# Autodesk Inventor assembly: CentralBeam1of2WithSails
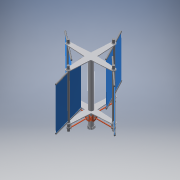
[picture p0: Inventor's stored thumbnail of the model, 180x180]
Saved by Autodesk Inventor 2016 SP1 (Build 200210100, 210)
## iProperties
Created: 2016-07-04
Part Number: CentralBeam1of2WithSails
Document SubType Name: Assembly
Designer: Tore Den Store
Author: Tore Den Store
## Documents named in this file (4)
- C:\Users\Jonatan\Documents\Inventor\Vertical axis wind turbine\WindPartCentral\CentralBeam1of2WithSails.iam
- C:\Users\Jonatan\Documents\Inventor\Vertical axis wind turbine\1 of 4 part\SailBeam.iam
- C:\Users\Jonatan\Documents\Inventor\Vertical axis wind turbine\WindPartCentral\WindCentralbeam.ipt
- C:\Users\Jonatan\Documents\Inventor\Vertical axis wind turbine\WindPartCentral\Connecting gears.ipt
## Components (9 placed, 3 different names)
1. SailBeam:1 [sub-assembly] — Rotational:1, Rotation:5
2. SailBeam:2 [sub-assembly] — Rotational:3, Rotation:2
3. SailBeam:3 [sub-assembly] — Rotational:4, Rotation:4
4. SailBeam:4 [sub-assembly] — Rotational:2, Rotation:1
5. WindCentralbeam:1 — Rotational:1, Rotational:2, Rotational:3, Rotational:4, Rotational:5, Rotational:6, Rotational:7, Rotational:8
6. Connecting gears:1 — Rotational:7, Rotation:2
7. Connecting gears:2 — Rotational:8, Rotation:1
8. Connecting gears:3 — Rotational:6, Rotation:5
9. Connecting gears:4 — Rotational:5, Rotation:4
## Relationships (12: RevoluteJoint 8, RelateRotation 4)
- Rotational:1 [RevoluteJoint]: SailBeam:1 ↔ WindCentralbeam:1
- Rotational:2 [RevoluteJoint]: SailBeam:4 ↔ WindCentralbeam:1
- Rotational:3 [RevoluteJoint]: SailBeam:2 ↔ WindCentralbeam:1
- Rotational:4 [RevoluteJoint]: SailBeam:3 ↔ WindCentralbeam:1
- Rotational:5 [RevoluteJoint]: WindCentralbeam:1 ↔ Connecting gears:4
- Rotational:6 [RevoluteJoint]: WindCentralbeam:1 ↔ Connecting gears:3
- Rotational:7 [RevoluteJoint]: WindCentralbeam:1 ↔ Connecting gears:1
- Rotational:8 [RevoluteJoint]: WindCentralbeam:1 ↔ Connecting gears:2
- Rotation:1 [RelateRotation] (0.25 ul): SailBeam:4 ↔ Connecting gears:2
- Rotation:2 [RelateRotation] (0.25 ul): SailBeam:2 ↔ Connecting gears:1
- Rotation:4 [RelateRotation] (0.25 ul): SailBeam:3 ↔ Connecting gears:4
- Rotation:5 [RelateRotation] (0.25 ul): SailBeam:1 ↔ Connecting gears:3
